# Autodesk Inventor assembly: two_wheels
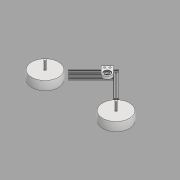
[picture p0: Inventor's stored thumbnail of the model, 180x180]
Saved by Autodesk Inventor 2021.3 (Build 253353000, 353)
## iProperties
Created: 2021-05-27
Part Number: two_wheels
Document SubType Name: Assembly
Designer: gisen
Author: gisen
## Documents named in this file (5)
- C:\Users\gisen\workspace\beetle_inventor_model\suspension\two_wheels.iam
- C:\Users\gisen\workspace\beetle_inventor_model\suspension\wheel_6inch_with_drum_brake.ipt
- C:\Users\gisen\workspace\beetle_inventor_model\suspension\AFS-2040-4-200.ipt
- C:\Users\gisen\workspace\beetle_inventor_model\suspension\AFS-2040-4-180.ipt
- C:\Users\gisen\workspace\beetle_inventor_model\suspension\SBGSMA6904ZZ-35\SBGSMA6904ZZ-35.iam
## Components (5 placed, 4 different names)
1. AFS-2040-4-200:1 — メイト:1, フラッシュ:1, フラッシュ:2, メイト:4, 対称度:1, フラッシュ:14
2. AFS-2040-4-180:1 — メイト:1, フラッシュ:1, フラッシュ:2, フラッシュ:4, メイト:2, 対称度:1
3. wheel_6inch_with_drum_brake:1 — フラッシュ:3, フラッシュ:4, メイト:2, メイト:9
4. wheel_6inch_with_drum_brake:2 — フラッシュ:3, メイト:4, メイト:8
5. SBGSMA6904ZZ-35:1 [sub-assembly]
## Relationships (20: Mate 13, Flush 5, Angle 1, Symmetry 1)
- メイト:1 [Mate]: AFS-2040-4-200:1 ↔ AFS-2040-4-180:1
- フラッシュ:1 [Flush]: AFS-2040-4-200:1 ↔ AFS-2040-4-180:1
- フラッシュ:2 [Flush]: AFS-2040-4-200:1 ↔ AFS-2040-4-180:1
- フラッシュ:3 [Flush]: wheel_6inch_with_drum_brake:1 ↔ wheel_6inch_with_drum_brake:2
- フラッシュ:4 [Flush]: AFS-2040-4-180:1 ↔ wheel_6inch_with_drum_brake:1
- メイト:2 [Mate]: AFS-2040-4-180:1 ↔ wheel_6inch_with_drum_brake:1
- メイト:4 [Mate]: AFS-2040-4-200:1 ↔ wheel_6inch_with_drum_brake:2
- [Mate]: AFS-2040-4-200:1 ↔ SBGSMA6904ZZ-35:1
- [Angle] (0 deg): AFS-2040-4-200:1 ↔ SBGSMA6904ZZ-35:1
- [Mate]: AFS-2040-4-200:1 ↔ SBGSMA6904ZZ-35:1
- 対称度:1 [Symmetry]: AFS-2040-4-200:1 ↔ AFS-2040-4-180:1
- [Mate]: SBGSMA6904ZZ-35:1
- メイト:8 [Mate]: wheel_6inch_with_drum_brake:2
- メイト:9 [Mate]: wheel_6inch_with_drum_brake:1
- メイト:10 [Mate]
- メイト:11 [Mate]
- メイト:12 [Mate]
- フラッシュ:14 [Flush]: AFS-2040-4-200:1
- メイト:13 [Mate]
- メイト:14 [Mate] (200 mm)
